# Autodesk Inventor assembly: Сальник 1
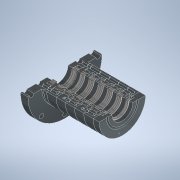
[picture p0: Inventor's stored thumbnail of the model, 180x180]
Saved by Autodesk Inventor 2021 (Build 250183000, 183)
## iProperties
Created: 2020-12-18
Part Number: Сальник 1
Document SubType Name: Assembly
Designer: Тимоха
Author: Тимоха
## Documents named in this file (15)
- C:\Users\Тимоха\Desktop\КР Компрессор\compressor\Сальник 1.iam
- C:\Users\Тимоха\Desktop\КР Компрессор\compressor\Корпус дросселя.ipt
- C:\Users\Тимоха\Desktop\КР Компрессор\compressor\Корпус сальника 1.ipt
- C:\Users\Тимоха\Desktop\КР Компрессор\compressor\Корпус сальника 2.ipt
- C:\Users\Тимоха\Desktop\КР Компрессор\compressor\Корпус сальника 3.ipt
- C:\Users\Тимоха\Desktop\КР Компрессор\compressor\Корпус сальника 4.ipt
- C:\Users\Тимоха\Desktop\КР Компрессор\compressor\Корпус сальника0.ipt
- C:\Users\Тимоха\Desktop\КР Компрессор\compressor\Крышка сальников.ipt
- C:\Users\Тимоха\Desktop\КР Компрессор\compressor\В сальник.ipt
- C:\Users\Тимоха\Desktop\КР Компрессор\compressor\Дроссельное кольцо.ipt
- C:\Users\Тимоха\Desktop\КР Компрессор\compressor\Кольцо сальника 1.ipt
- C:\Users\Тимоха\Desktop\КР Компрессор\compressor\Кольцо сальника 2.ipt
- C:\Users\Тимоха\Desktop\КР Компрессор\compressor\Кольцо сальника.ipt
- C:\Users\Тимоха\Desktop\КР Компрессор\compressor\Пружина дросселя.ipt
- C:\Users\Тимоха\Desktop\КР Компрессор\compressor\Пружина сальника.ipt
## Components (46 placed, 14 different names)
1. Корпус дросселя:1 — Жесткий:39
2. Корпус сальника 1:1 — Жесткий:41
3. Корпус сальника 2:1 — Жесткий:42
4. Корпус сальника 3:1 — Жесткий:43
5. Корпус сальника 4:1 — Жесткий:44
6. Корпус сальника0:1 — Жесткий:40
7. Крышка сальников:1 — Жесткий:45
8. В сальник:1
9. Дроссельное кольцо:1 — Жесткий:11, Жесткий:39
10. Кольцо сальника 1:1 — Жесткий:10, Жесткий:17, Жесткий:18
11. Кольцо сальника 2:1 — Жесткий:9, Жесткий:17
12. Кольцо сальника:1 — Жесткий:8, Жесткий:18, Жесткий:44
13. Пружина дросселя:1 — Жесткий:11
14. Пружина сальника:1 — Жесткий:10
15. Пружина сальника:2 — Жесткий:8
16. Пружина сальника:3 — Жесткий:9
17. Кольцо сальника:2 — Жесткий:15
18. Пружина сальника:4
19. Кольцо сальника:3 — Жесткий:15, Жесткий:16
20. Пружина сальника:5
21. Кольцо сальника:4 — Жесткий:16, Жесткий:40
22. Пружина сальника:6
23. Кольцо сальника 1:2
24. Кольцо сальника 2:2
25. Кольцо сальника:5 — Жесткий:45
26. Пружина сальника:7
27. Пружина сальника:8
28. Пружина сальника:9
29. Кольцо сальника:6
30. Пружина сальника:10
31. Кольцо сальника:7
32. Пружина сальника:11
33. Кольцо сальника:8 — Жесткий:42
34. Пружина сальника:12
35. Кольцо сальника:9
36. Пружина сальника:13
37. Кольцо сальника:10
38. Пружина сальника:14
39. Кольцо сальника:11 — Жесткий:43
40. Пружина сальника:15
41. Кольцо сальника:12
42. Пружина сальника:16
43. Кольцо сальника:13
44. Пружина сальника:17
45. Кольцо сальника:14 — Жесткий:41
46. Пружина сальника:18
## Relationships (45: WeldJoint 45)
- [WeldJoint]: Корпус дросселя:1 ↔ Корпус сальника0:1
- [WeldJoint]: Корпус сальника 1:1 ↔ Корпус сальника0:1
- [WeldJoint]: Корпус сальника 1:1 ↔ Корпус сальника 2:1
- [WeldJoint]: Корпус сальника 2:1 ↔ Корпус сальника 3:1
- [WeldJoint]: Корпус сальника 3:1 ↔ Корпус сальника 4:1
- [WeldJoint]: Корпус сальника 4:1 ↔ В сальник:1
- [WeldJoint]: Крышка сальников:1 ↔ В сальник:1
- Жесткий:8 [WeldJoint]: Кольцо сальника:1 ↔ Пружина сальника:2
- Жесткий:9 [WeldJoint]: Кольцо сальника 2:1 ↔ Пружина сальника:3
- Жесткий:10 [WeldJoint]: Кольцо сальника 1:1 ↔ Пружина сальника:1
- Жесткий:11 [WeldJoint]: Дроссельное кольцо:1 ↔ Пружина дросселя:1
- [WeldJoint]: Кольцо сальника:2 ↔ Пружина сальника:4
- [WeldJoint]: Кольцо сальника:3 ↔ Пружина сальника:5
- [WeldJoint]: Кольцо сальника:4 ↔ Пружина сальника:6
- Жесткий:15 [WeldJoint]: Кольцо сальника:2 ↔ Кольцо сальника:3
- Жесткий:16 [WeldJoint]: Кольцо сальника:3 ↔ Кольцо сальника:4
- Жесткий:17 [WeldJoint]: Кольцо сальника 1:1 ↔ Кольцо сальника 2:1
- Жесткий:18 [WeldJoint]: Кольцо сальника 1:1 ↔ Кольцо сальника:1
- [WeldJoint]: Кольцо сальника:5 ↔ Пружина сальника:8
- [WeldJoint]: Кольцо сальника 2:2 ↔ Пружина сальника:9
- [WeldJoint]: Кольцо сальника 1:2 ↔ Пружина сальника:7
- [WeldJoint]: Кольцо сальника 1:2 ↔ Кольцо сальника 2:2
- [WeldJoint]: Кольцо сальника 1:2 ↔ Кольцо сальника:5
- [WeldJoint]: Кольцо сальника:6 ↔ Пружина сальника:10
- [WeldJoint]: Кольцо сальника:7 ↔ Пружина сальника:11
- [WeldJoint]: Кольцо сальника:8 ↔ Пружина сальника:12
- [WeldJoint]: Кольцо сальника:6 ↔ Кольцо сальника:7
- [WeldJoint]: Кольцо сальника:7 ↔ Кольцо сальника:8
- [WeldJoint]: Кольцо сальника:9 ↔ Пружина сальника:13
- [WeldJoint]: Кольцо сальника:10 ↔ Пружина сальника:14
- [WeldJoint]: Кольцо сальника:11 ↔ Пружина сальника:15
- [WeldJoint]: Кольцо сальника:9 ↔ Кольцо сальника:10
- [WeldJoint]: Кольцо сальника:10 ↔ Кольцо сальника:11
- [WeldJoint]: Кольцо сальника:12 ↔ Пружина сальника:16
- [WeldJoint]: Кольцо сальника:13 ↔ Пружина сальника:17
- [WeldJoint]: Кольцо сальника:14 ↔ Пружина сальника:18
- [WeldJoint]: Кольцо сальника:12 ↔ Кольцо сальника:13
- [WeldJoint]: Кольцо сальника:13 ↔ Кольцо сальника:14
- Жесткий:39 [WeldJoint]: Корпус дросселя:1 ↔ Дроссельное кольцо:1
- Жесткий:40 [WeldJoint]: Корпус сальника0:1 ↔ Кольцо сальника:4
- Жесткий:41 [WeldJoint]: Корпус сальника 1:1 ↔ Кольцо сальника:14
- Жесткий:42 [WeldJoint]: Корпус сальника 2:1 ↔ Кольцо сальника:8
- Жесткий:43 [WeldJoint]: Корпус сальника 3:1 ↔ Кольцо сальника:11
- Жесткий:44 [WeldJoint]: Корпус сальника 4:1 ↔ Кольцо сальника:1
- Жесткий:45 [WeldJoint]: Крышка сальников:1 ↔ Кольцо сальника:5
## Named parameters: d11_d7 = 0 mm, d12_d7 = 0 mm, d13_d7 = 0 mm, d18_d7 = 0 mm, d19_d8 = 0 mm, d20_d9 = 0 mm, d21_d16 = 0 mm, d22_d17 = 0 mm, d23_d11_d7 = 0 mm, d24_d12_d7 = 0 mm, d25_d13_d7 = 0 mm, d26_d14 = 0 mm, d27_d15 = 0 mm, d28_d11_d7 = 0 mm, d29_d12_d7 = 0 mm, d30_d13_d7 = 0 mm, d31_d14 = 0 mm, d32_d15 = 0 mm, d33_d11_d7 = 0 mm, d34_d12_d7 = 0 mm, d35_d13_d7 = 0 mm, d36_d14 = 0 mm, d37_d15 = 0 mm
